# Autodesk Inventor assembly: corner
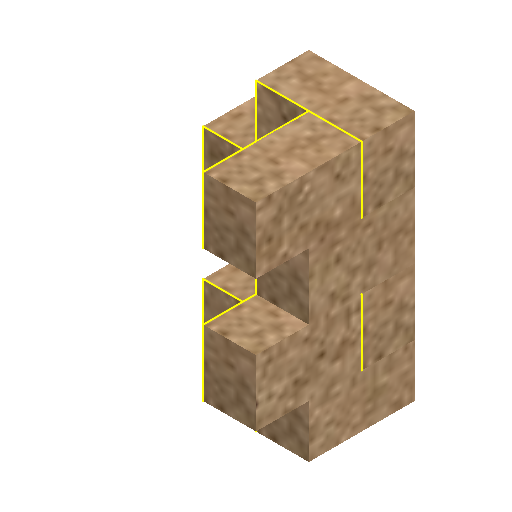
[picture p0: Inventor's stored thumbnail of the model, 512x512]
Saved by Autodesk Inventor 2025 (Build 290162000, 162)
## iProperties
Created: 2024-09-26
Part Number: corner
Document SubType Name: Assembly
Designer: DANIEL
Author: DANIEL
## Documents named in this file (2)
- C:\Users\DANIEL\Documents\EIA\Semestres\08\RoboticaIndustrial\labs\06\DIFFCAR_CAD\corner.iam
- C:\Users\DANIEL\Documents\EIA\Semestres\08\RoboticaIndustrial\labs\06\DIFFCAR_CAD\wall2.ipt
## Components (2 placed, 1 different names)
1. wall2:1 — Mate:1, Mate:2, Mate:3
2. wall2:2 — Mate:1, Mate:2, Mate:3
## Relationships (3: Mate 3)
- Mate:1: wall2:1 ↔ wall2:2
- Mate:2: wall2:1 ↔ wall2:2
- Mate:3: wall2:1 ↔ wall2:2
